# Autodesk Inventor assembly: Drive Wheel Assembly with Perf Wheels
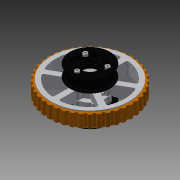
[picture p0: Inventor's stored thumbnail of the model, 180x180]
Saved by Autodesk Inventor 2013 (Build 170138000, 138)
## iProperties
Created: 2013-02-07
Part Number: Drive Wheel Assembly with Perf Wheels
Document SubType Name: Assembly
Designer: Moses
Author: Moses
## Documents named in this file (6)
- C:\Users\Moses\Documents\GitHub\frc2013CAD\Drivetrain\Drive Wheel Assembly with Perf Wheels.iam
- C:\Users\Moses\Documents\GitHub\frc2013CAD\Drivetrain\6 Perf ThruTread 500 Hex\6 Perf Plaction Tread 500 Hex.iam
- C:\Users\Moses\Documents\GitHub\frc2013CAD\Drivetrain\DBK_42ToothPulley (am-2234)\DBK_42ToothPulley V2.iam
- C:\Users\Moses\Documents\GitHub\frc2013CAD\Drivetrain\Custom Belt Pulley Hex Hub.ipt
- C:\Users\Moses\Documents\GitHub\frc2013CAD\Drivetrain\91251A980 10-24 Screw\91251A980.ipt
- C:\Users\Moses\Documents\GitHub\frc2013CAD\Drivetrain\Custom Belt Pulley Hex Hub (polycarbonate).ipt
## Components (10 placed, 5 different names)
1. 6 Perf Plaction Tread 500 Hex:1 [sub-assembly] — Mate:7, Mate:8, Mate:9, Mate:10, Mate:11, Mate:18
2. DBK_42ToothPulley V2:1 [sub-assembly] — Mate:10, Mate:11, Insert:1, Insert:2, Insert:3, Mate:12, Mate:14
3. DBK_42ToothPulley V2:2 [sub-assembly] — Mate:2, Mate:3, Mate:8, Mate:9, Mate:1, Mate:15, Mate:16
4. Custom Belt Pulley Hex Hub:1 — Mate:2, Mate:3, Mate:4, Mate:5, Mate:6, Mate:17
5. Custom Belt Pulley Hex Hub:2 — Mate:4, Mate:5, Mate:6, Mate:7
6. 91251A980:1 — Insert:2
7. 91251A980:2 — Insert:3
8. 91251A980:3 — Insert:1, Mate:13
9. Custom Belt Pulley Hex Hub (polycarbonate):1 — Mate:12, Mate:13, Mate:14, Mate:18
10. Custom Belt Pulley Hex Hub (polycarbonate):2 — Mate:1, Mate:15, Mate:16, Mate:17
## Relationships (21: Mate 18, Insert 3)
- Mate:1: DBK_42ToothPulley V2:2 ↔ Custom Belt Pulley Hex Hub (polycarbonate):2
- Mate:2: DBK_42ToothPulley V2:2 ↔ Custom Belt Pulley Hex Hub:1
- Mate:3: DBK_42ToothPulley V2:2 ↔ Custom Belt Pulley Hex Hub:1
- Mate:4: Custom Belt Pulley Hex Hub:1 ↔ Custom Belt Pulley Hex Hub:2
- Mate:5: Custom Belt Pulley Hex Hub:1 ↔ Custom Belt Pulley Hex Hub:2
- Mate:6: Custom Belt Pulley Hex Hub:1 ↔ Custom Belt Pulley Hex Hub:2
- Mate:7: 6 Perf Plaction Tread 500 Hex:1 ↔ Custom Belt Pulley Hex Hub:2
- Mate:8: 6 Perf Plaction Tread 500 Hex:1 ↔ DBK_42ToothPulley V2:2
- Mate:9: 6 Perf Plaction Tread 500 Hex:1 ↔ DBK_42ToothPulley V2:2
- Mate:10: 6 Perf Plaction Tread 500 Hex:1 ↔ DBK_42ToothPulley V2:1
- Mate:11: 6 Perf Plaction Tread 500 Hex:1 ↔ DBK_42ToothPulley V2:1
- Insert:1: DBK_42ToothPulley V2:1 ↔ 91251A980:3
- Insert:2: DBK_42ToothPulley V2:1 ↔ 91251A980:1
- Insert:3: DBK_42ToothPulley V2:1 ↔ 91251A980:2
- Mate:12: DBK_42ToothPulley V2:1 ↔ Custom Belt Pulley Hex Hub (polycarbonate):1
- Mate:13: 91251A980:3 ↔ Custom Belt Pulley Hex Hub (polycarbonate):1
- Mate:14: DBK_42ToothPulley V2:1 ↔ Custom Belt Pulley Hex Hub (polycarbonate):1
- Mate:15: DBK_42ToothPulley V2:2 ↔ Custom Belt Pulley Hex Hub (polycarbonate):2
- Mate:16: DBK_42ToothPulley V2:2 ↔ Custom Belt Pulley Hex Hub (polycarbonate):2
- Mate:17: Custom Belt Pulley Hex Hub:1 ↔ Custom Belt Pulley Hex Hub (polycarbonate):2
- Mate:18: 6 Perf Plaction Tread 500 Hex:1 ↔ Custom Belt Pulley Hex Hub (polycarbonate):1
